# Autodesk Inventor assembly: Case Bottom
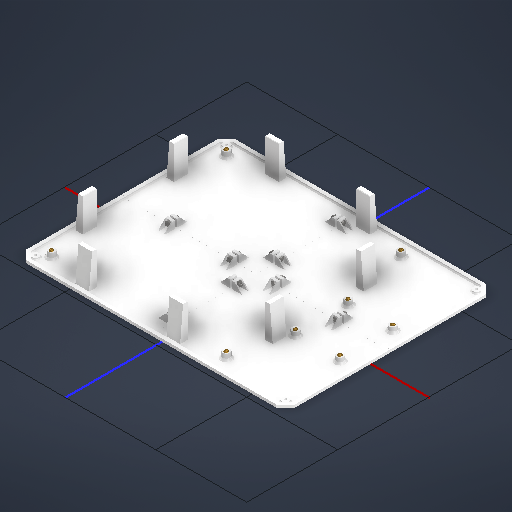
[picture p0: Inventor's stored thumbnail of the model, 512x512]
Saved by Autodesk Inventor 2026 (Build 300175000, 175)
## iProperties
Created: 2025-06-13
Part Number: Case Bottom
Document SubType Name: Assembly
Designer: ckyiu
Author: ckyiu
## Documents named in this file (8)
- C:\Users\ckyiu\Documents\Projects\Chessboard-Design\Design\Case\Case Bottom.iam
- C:\Users\ckyiu\Documents\Projects\Chessboard-Design\Design\Case\Case Bottom BR.ipt
- C:\Users\ckyiu\Documents\Projects\Chessboard-Design\Design\Case\Case Bottom TL.ipt
- C:\Users\ckyiu\Documents\Projects\Chessboard-Design\Design\Case\Case Bottom TR.ipt
- C:\Users\ckyiu\Documents\Projects\Chessboard-Design\Design\Case\Case Bottom BL.ipt
- C:\Users\ckyiu\Documents\Projects\Chessboard-Design\Design\Hardware\M2.5\Heat set inserts\(4mm) 94459A768_Heat-Set Inserts for Plastic.ipt
- C:\Users\ckyiu\Documents\Projects\Chessboard-Design\Design\Hardware\M2.5\Screws\(12mm) 92000A107_Passivated 18-8 Stainless Steel Pan Head Phillips Screws.ipt
- C:\Users\ckyiu\Documents\Projects\Chessboard-Design\Design\Hardware\M2.5\Nuts\(2mm) 91828A113_18-8 Stainless Steel Hex Nut.ipt
## Components (28 placed, 7 different names)
1. Case Bottom BR:1 — Mate:3, Mate:4, Flush:3, Flush:4, Flush:6, Flush:7, Insert:3, Insert:7, Insert:8, Insert:9, Insert:10, Insert:19, Insert:20
2. Case Bottom TL:1 — Mate:1, Mate:2, Flush:1, Flush:2, Flush:5, Flush:8, Insert:2, Insert:13, Insert:14, Insert:23, Insert:24
3. Case Bottom TR:1 — Mate:2, Mate:4, Flush:2, Flush:4, Flush:5, Flush:6, Insert:4, Insert:5, Insert:6, Insert:11, Insert:12, Insert:21, Insert:22
4. Case Bottom BL:1 — Mate:1, Mate:3, Flush:1, Flush:3, Flush:7, Flush:8, Insert:1, Insert:15, Insert:16, Insert:17, Insert:18
5. (4mm) 94459A768_Heat-Set Inserts for Plastic:1 — Insert:1
6. (4mm) 94459A768_Heat-Set Inserts for Plastic:2 — Insert:4
7. (4mm) 94459A768_Heat-Set Inserts for Plastic:3 — Insert:3
8. (4mm) 94459A768_Heat-Set Inserts for Plastic:4 — Insert:2
9. (4mm) 94459A768_Heat-Set Inserts for Plastic:5 — Insert:5
10. (4mm) 94459A768_Heat-Set Inserts for Plastic:6 — Insert:7
11. (4mm) 94459A768_Heat-Set Inserts for Plastic:7 — Insert:8
12. (4mm) 94459A768_Heat-Set Inserts for Plastic:8 — Insert:6
13. (12mm) 92000A107_Passivated 18-8 Stainless Steel Pan Head Phillips Screws:1 — Insert:9
14. (12mm) 92000A107_Passivated 18-8 Stainless Steel Pan Head Phillips Screws:2 — Insert:10
15. (12mm) 92000A107_Passivated 18-8 Stainless Steel Pan Head Phillips Screws:3 — Insert:11
16. (12mm) 92000A107_Passivated 18-8 Stainless Steel Pan Head Phillips Screws:4 — Insert:12
17. (12mm) 92000A107_Passivated 18-8 Stainless Steel Pan Head Phillips Screws:5 — Insert:13
18. (12mm) 92000A107_Passivated 18-8 Stainless Steel Pan Head Phillips Screws:6 — Insert:14
19. (12mm) 92000A107_Passivated 18-8 Stainless Steel Pan Head Phillips Screws:7 — Insert:15
20. (12mm) 92000A107_Passivated 18-8 Stainless Steel Pan Head Phillips Screws:8 — Insert:16
21. (2mm) 91828A113_18-8 Stainless Steel Hex Nut:1 — Insert:17
22. (2mm) 91828A113_18-8 Stainless Steel Hex Nut:2 — Insert:18
23. (2mm) 91828A113_18-8 Stainless Steel Hex Nut:3 — Insert:23
24. (2mm) 91828A113_18-8 Stainless Steel Hex Nut:4 — Insert:21
25. (2mm) 91828A113_18-8 Stainless Steel Hex Nut:5 — Insert:22
26. (2mm) 91828A113_18-8 Stainless Steel Hex Nut:6 — Insert:24
27. (2mm) 91828A113_18-8 Stainless Steel Hex Nut:7 — Insert:19
28. (2mm) 91828A113_18-8 Stainless Steel Hex Nut:8 — Insert:20
## Relationships (36: Insert 24, Flush 8, Mate 4)
- Mate:1: Case Bottom TL:1 ↔ Case Bottom BL:1
- Mate:2: Case Bottom TL:1 ↔ Case Bottom TR:1
- Mate:3: Case Bottom BR:1 ↔ Case Bottom BL:1
- Mate:4: Case Bottom BR:1 ↔ Case Bottom TR:1
- Flush:1: Case Bottom TL:1 ↔ Case Bottom BL:1
- Flush:2: Case Bottom TL:1 ↔ Case Bottom TR:1
- Flush:3: Case Bottom BR:1 ↔ Case Bottom BL:1
- Flush:4: Case Bottom BR:1 ↔ Case Bottom TR:1
- Flush:5: Case Bottom TL:1 ↔ Case Bottom TR:1
- Flush:6: Case Bottom BR:1 ↔ Case Bottom TR:1
- Flush:7: Case Bottom BR:1 ↔ Case Bottom BL:1
- Flush:8: Case Bottom TL:1 ↔ Case Bottom BL:1
- Insert:1 (-0.01 mm): Case Bottom BL:1 ↔ (4mm) 94459A768_Heat-Set Inserts for Plastic:1
- Insert:2 (-0.01 mm): Case Bottom TL:1 ↔ (4mm) 94459A768_Heat-Set Inserts for Plastic:4
- Insert:3 (-0.01 mm): Case Bottom BR:1 ↔ (4mm) 94459A768_Heat-Set Inserts for Plastic:3
- Insert:4 (-0.01 mm): Case Bottom TR:1 ↔ (4mm) 94459A768_Heat-Set Inserts for Plastic:2
- Insert:5 (-0.01 mm): Case Bottom TR:1 ↔ (4mm) 94459A768_Heat-Set Inserts for Plastic:5
- Insert:6 (-0.01 mm): Case Bottom TR:1 ↔ (4mm) 94459A768_Heat-Set Inserts for Plastic:8
- Insert:7 (-0.01 mm): Case Bottom BR:1 ↔ (4mm) 94459A768_Heat-Set Inserts for Plastic:6
- Insert:8 (-0.01 mm): Case Bottom BR:1 ↔ (4mm) 94459A768_Heat-Set Inserts for Plastic:7
- Insert:9: Case Bottom BR:1 ↔ (12mm) 92000A107_Passivated 18-8 Stainless Steel Pan Head Phillips Screws:1
- Insert:10: Case Bottom BR:1 ↔ (12mm) 92000A107_Passivated 18-8 Stainless Steel Pan Head Phillips Screws:2
- Insert:11: Case Bottom TR:1 ↔ (12mm) 92000A107_Passivated 18-8 Stainless Steel Pan Head Phillips Screws:3
- Insert:12: Case Bottom TR:1 ↔ (12mm) 92000A107_Passivated 18-8 Stainless Steel Pan Head Phillips Screws:4
- Insert:13: Case Bottom TL:1 ↔ (12mm) 92000A107_Passivated 18-8 Stainless Steel Pan Head Phillips Screws:5
- Insert:14: Case Bottom TL:1 ↔ (12mm) 92000A107_Passivated 18-8 Stainless Steel Pan Head Phillips Screws:6
- Insert:15: Case Bottom BL:1 ↔ (12mm) 92000A107_Passivated 18-8 Stainless Steel Pan Head Phillips Screws:7
- Insert:16: Case Bottom BL:1 ↔ (12mm) 92000A107_Passivated 18-8 Stainless Steel Pan Head Phillips Screws:8
- Insert:17: Case Bottom BL:1 ↔ (2mm) 91828A113_18-8 Stainless Steel Hex Nut:1
- Insert:18: Case Bottom BL:1 ↔ (2mm) 91828A113_18-8 Stainless Steel Hex Nut:2
- Insert:19: Case Bottom BR:1 ↔ (2mm) 91828A113_18-8 Stainless Steel Hex Nut:7
- Insert:20: Case Bottom BR:1 ↔ (2mm) 91828A113_18-8 Stainless Steel Hex Nut:8
- Insert:21: Case Bottom TR:1 ↔ (2mm) 91828A113_18-8 Stainless Steel Hex Nut:4
- Insert:22: Case Bottom TR:1 ↔ (2mm) 91828A113_18-8 Stainless Steel Hex Nut:5
- Insert:23: Case Bottom TL:1 ↔ (2mm) 91828A113_18-8 Stainless Steel Hex Nut:3
- Insert:24: Case Bottom TL:1 ↔ (2mm) 91828A113_18-8 Stainless Steel Hex Nut:6
